# Autodesk Inventor assembly: inner_body
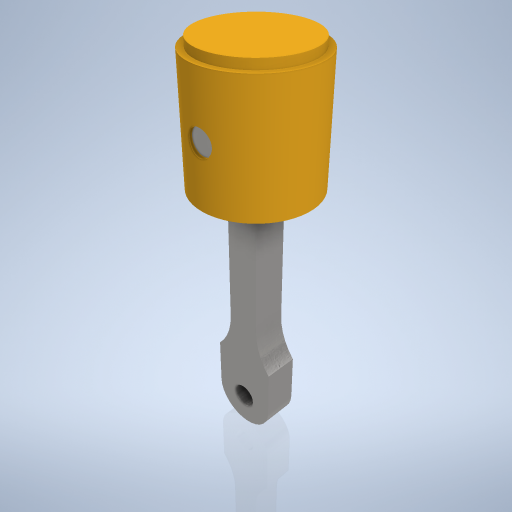
[picture p0: Inventor's stored thumbnail of the model, 512x512]
Saved by Autodesk Inventor 2024.2 (Build 282272000, 272)
## iProperties
Created: 2024-04-07
Part Number: inner_body
Document SubType Name: Assembly
Designer: Fabri
Author: Fabri
## Documents named in this file (4)
- C:\Users\Fabri\Documents\Inventor\Durckluft\inner_body.iam
- C:\Users\Fabri\Documents\Inventor\Durckluft\Pleuel.ipt
- C:\Users\Fabri\Documents\Inventor\Durckluft\Kolben.ipt
- C:\Users\Fabri\Documents\Inventor\Durckluft\Kurbelzapfen.ipt
## Components (3 placed, 3 different names)
1. Kurbelzapfen:1 — Einfügen:1, Drehbar:1
2. Kolben:1 — Drehbar:1
3. Pleuel:1 — Einfügen:1
## Relationships (2: Insert 1, RevoluteJoint 1)
- Einfügen:1 [Insert] (-8.5 mm): Kurbelzapfen:1 ↔ Pleuel:1
- Drehbar:1 [RevoluteJoint] (2 mm): Kurbelzapfen:1 ↔ Kolben:1
